# Autodesk Inventor assembly: Conjunto Superior
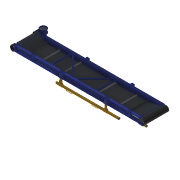
[picture p0: Inventor's stored thumbnail of the model, 180x180]
Saved by Autodesk Inventor 2019 (Build 230136000, 136)
## iProperties
Created: 2020-02-06
Part Number: Conjunto Superior
Document SubType Name: Assembly
Designer: Juan Carlos Botero
Author: Juan Carlos Botero
## Documents named in this file (5)
- D:\Drives\OneDrive\Carlos_2\02 TRABAJOS\MULTIPLO\Conveyor\ENSAMBLE\Conjunto Superior.iam
- D:\Drives\OneDrive\Carlos_2\02 TRABAJOS\MULTIPLO\Conveyor\ENSAMBLE\Bumpers.iam
- D:\Drives\OneDrive\Carlos_2\02 TRABAJOS\MULTIPLO\Conveyor\ENSAMBLE\Banda.iam
- D:\Drives\OneDrive\Carlos_2\02 TRABAJOS\MULTIPLO\Conveyor\ENSAMBLE\Botonera 3 botones _2_.iam
- D:\Drives\OneDrive\Carlos_2\02 TRABAJOS\MULTIPLO\Conveyor\ENSAMBLE\Botón de emergencia _2_.iam
## Components (6 placed, 4 different names)
1. Bumpers:1 [sub-assembly]
2. Banda:1 [sub-assembly] — Rotational:1, Mate:1, Mate:2, Mate:3, Rigid:1, Mate:4, Mate:5, Angle:1
3. Botonera 3 botones _2_:1 [sub-assembly] — Mate:1, Mate:2, Mate:3
4. Botón de emergencia _2_:1 [sub-assembly] — Rotational:1
5. Botonera 3 botones _2_:2 [sub-assembly] — Mate:4, Mate:5, Angle:1
6. Botón de emergencia _2_:2 [sub-assembly] — Rigid:1
## Relationships (8: Mate 5, RevoluteJoint 1, WeldJoint 1, Angle 1)
- Rotational:1 [RevoluteJoint]: Banda:1 ↔ Botón de emergencia _2_:1
- Mate:1: Banda:1 ↔ Botonera 3 botones _2_:1
- Mate:2: Banda:1 ↔ Botonera 3 botones _2_:1
- Mate:3 (50 mm): Banda:1 ↔ Botonera 3 botones _2_:1
- Rigid:1 [WeldJoint]: Banda:1 ↔ Botón de emergencia _2_:2
- Mate:4: Banda:1 ↔ Botonera 3 botones _2_:2
- Mate:5: Banda:1 ↔ Botonera 3 botones _2_:2
- Angle:1 (90 deg): Banda:1 ↔ Botonera 3 botones _2_:2
